# Autodesk Inventor assembly: arm_MIR
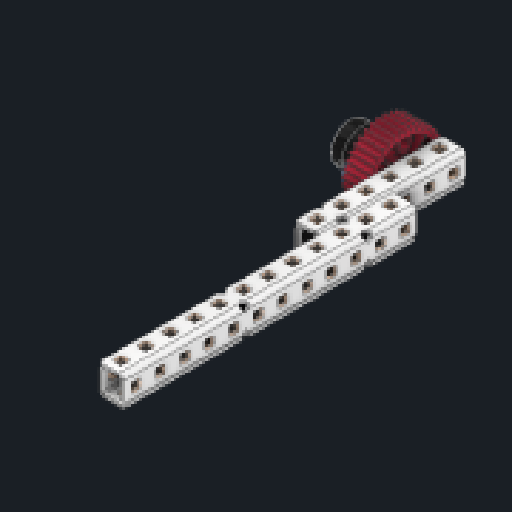
[picture p0: Inventor's stored thumbnail of the model, 512x512]
Saved by Autodesk Inventor 2024 (Build 280153000, 153)
## iProperties
Created: 2023-08-16
Part Number: arm_MIR
Document SubType Name: Assembly
Designer: avere
Author: avere
## Documents named in this file (10)
- D:\vex_robotics\hardware\cad\scrap_v0.1\catapult\mirrored_parts\arm_MIR.iam
- D:\vex_robotics\hardware\cad\VEX-CAD-Inventor-1.41\Motion\Spacers\Spacer Nylon .375 OD\NSpacer .375 OD x .375.ipt
- D:\vex_robotics\hardware\cad\VEX-CAD-Inventor-1.41\Motion\Spacers\Spacer Nylon .375 OD.ipt
- D:\vex_robotics\hardware\cad\scrap_v0.1\catapult\mirrored_parts\HS 36T Gear, No Insert_MIR.iam
- D:\vex_robotics\hardware\cad\scrap_v0.1\catapult\mirrored_parts\Alu Angle 1x1x6_MIR.ipt
- D:\vex_robotics\hardware\cad\VEX-CAD-Inventor-1.41\Motion\Shaft HS\HS Spacer.ipt
- D:\vex_robotics\hardware\cad\VEX-CAD-Inventor-1.41\Motion\Shaft HS\HS Shaft Collar.ipt
- D:\vex_robotics\hardware\cad\VEX-CAD-Inventor-1.41\Structure\Hardware\Nut Hex.ipt
- D:\vex_robotics\hardware\cad\VEX-CAD-Inventor-1.41\Motion\Shaft HS\HS Spacer\HSpacer .1250.ipt
- D:\vex_robotics\hardware\cad\VEX-CAD-Inventor-1.41\Structure\Angle\Aluminum 1x1\Alu Angle 1x1x12.ipt
## Components (14 placed, 7 different names)
1. NSpacer .375 OD x .375:1 — Insert:19, Insert:20
2. HS 36T Gear, No Insert_MIR:1 [sub-assembly] — Mate:2, Insert:11, Insert:12, Insert:13, Insert:14
3. NSpacer .375 OD x .375:2 — Insert:18, Mate:4
4. Alu Angle 1x1x6_MIR:1 — Mate:2, Insert:11, Insert:7, Insert:9, Insert:16
5. Alu Angle 1x1x6_MIR:2 — Insert:8, Insert:10, Insert:17, Mate:3
6. NSpacer .375 OD x .375:3 — Insert:8, Insert:7
7. NSpacer .375 OD x .375:4 — Insert:10, Insert:9
8. HS Shaft Collar:1 — Insert:15
9. Nut Hex:1 — Insert:12
10. Nut Hex:2 — Insert:13
11. HSpacer .1250:1 — Insert:14, Insert:15
12. NSpacer .375 OD x .375:5 — Insert:16
13. Alu Angle 1x1x12:1 — Insert:17, Mate:3, Insert:18, Insert:19
14. Alu Angle 1x1x12:2 — Insert:20, Mate:4
## Relationships (17: Insert 14, Mate 3)
- Mate:2: HS 36T Gear, No Insert_MIR:1 ↔ Alu Angle 1x1x6_MIR:1
- Insert:11: HS 36T Gear, No Insert_MIR:1 ↔ Alu Angle 1x1x6_MIR:1
- Insert:8: Alu Angle 1x1x6_MIR:2 ↔ NSpacer .375 OD x .375:3
- Insert:7: Alu Angle 1x1x6_MIR:1 ↔ NSpacer .375 OD x .375:3
- Insert:10: Alu Angle 1x1x6_MIR:2 ↔ NSpacer .375 OD x .375:4
- Insert:9: Alu Angle 1x1x6_MIR:1 ↔ NSpacer .375 OD x .375:4
- Insert:12: HS 36T Gear, No Insert_MIR:1 ↔ Nut Hex:1
- Insert:13: HS 36T Gear, No Insert_MIR:1 ↔ Nut Hex:2
- Insert:14: HS 36T Gear, No Insert_MIR:1 ↔ HSpacer .1250:1
- Insert:15: HS Shaft Collar:1 ↔ HSpacer .1250:1
- Insert:16: Alu Angle 1x1x6_MIR:1 ↔ NSpacer .375 OD x .375:5
- Insert:17: Alu Angle 1x1x6_MIR:2 ↔ Alu Angle 1x1x12:1
- Mate:3: Alu Angle 1x1x6_MIR:2 ↔ Alu Angle 1x1x12:1
- Insert:18: NSpacer .375 OD x .375:2 ↔ Alu Angle 1x1x12:1
- Insert:19: NSpacer .375 OD x .375:1 ↔ Alu Angle 1x1x12:1
- Insert:20: NSpacer .375 OD x .375:1 ↔ Alu Angle 1x1x12:2
- Mate:4: NSpacer .375 OD x .375:2 ↔ Alu Angle 1x1x12:2
